# Autodesk Inventor assembly: 211-03
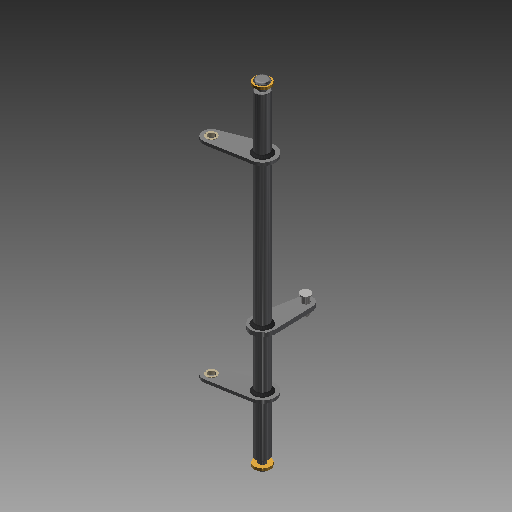
[picture p0: Inventor's stored thumbnail of the model, 512x512]
Saved by Autodesk Inventor 2019 (Build 230136000, 136)
## iProperties
Company: Autodesk Inc.
Created: 2007-12-25
Part Number: 211-03
Document SubType Name: Assembly
Designer: Autodesk Inc.
Mass: 762.491 g
Surface Area: 385.153 cm^2
Volume: 97.3313 cm^3
Density: 7.83397 g/cm^3
Description: PIVOT LINK WELDMENT
Component Category: Lower Component
Author: Inventor
## Documents named in this file (5)
- C:\TEMP\Car Seat\Workspace\Pivot Link Weldment.iam
- C:\TEMP\Car Seat\Workspace\Rear Pivot Link Weldment.iam
- C:\TEMP\Car Seat\Workspace\Bushing 2.ipt
- C:\TEMP\Car Seat\Workspace\Brass Spacer.ipt
- C:\TEMP\Car Seat\Workspace\Rear Pivot Pin.ipt
## Components (6 placed, 4 different names)
1. Rear Pivot Link Weldment:1 [sub-assembly] — Insert:1, Insert:2, Angle:1, Angle:2, Insert:3, Insert:4, Insert:5
2. Bushing 2:2 — Insert:1, Angle:2
3. Bushing 2:1 — Insert:2, Angle:1
4. Brass Spacer:1 — Insert:3
5. Brass Spacer:2 — Insert:4
6. Rear Pivot Pin:1 — Insert:5
## Relationships (7: Insert 5, Angle 2)
- Insert:1: Rear Pivot Link Weldment:1 ↔ Bushing 2:2
- Insert:2: Rear Pivot Link Weldment:1 ↔ Bushing 2:1
- Angle:1 (0 deg): Rear Pivot Link Weldment:1 ↔ Bushing 2:1
- Angle:2 (0 deg): Rear Pivot Link Weldment:1 ↔ Bushing 2:2
- Insert:3: Rear Pivot Link Weldment:1 ↔ Brass Spacer:1
- Insert:4: Rear Pivot Link Weldment:1 ↔ Brass Spacer:2
- Insert:5 (7.5 mm): Rear Pivot Link Weldment:1 ↔ Rear Pivot Pin:1
